# Autodesk Inventor assembly: BC-100001_B
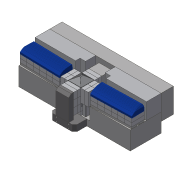
[picture p0: Inventor's stored thumbnail of the model, 180x180]
Saved by Autodesk Inventor 2016 (Build 200138000, 138)
## iProperties
Created: 2015-09-16
Part Number: BC-100001_B
Document SubType Name: Assembly
Designer: Reinaldo.Basílio
Author: Reinaldo.Basílio
## Documents named in this file (25)
- D:\ARQ\Basilio\LNLS-2\Anel\Dipolos\BC-3T\Dipolo 3T e 1T\Prototipo 1\Desenhos\BC-100001_B.iam
- D:\ARQ\Basilio\LNLS-2\Anel\Dipolos\BC-3T\Dipolo 3T e 1T\Prototipo 1\Desenhos\BC-100003.iam
- D:\ARQ\Basilio\LNLS-2\Anel\Dipolos\BC-3T\Dipolo 3T e 1T\Prototipo 1\Desenhos\BC-100004.iam
- D:\ARQ\Basilio\LNLS-2\Anel\Dipolos\BC-3T\Dipolo 3T e 1T\Prototipo 1\Desenhos\BC-10009.ipt
- D:\ARQ\Basilio\LNLS-2\Anel\Dipolos\BC-3T\Dipolo 3T e 1T\Prototipo 1\Desenhos\BC-100005.iam
- D:\ARQ\Basilio\LNLS-2\Anel\Dipolos\BC-3T\Dipolo 3T e 1T\Prototipo 1\Desenhos\BC-10010.ipt
- D:\ARQ\Basilio\LNLS-2\Anel\Dipolos\BC-3T\Dipolo 3T e 1T\Prototipo 1\Desenhos\BC-10011.ipt
- D:\ARQ\Basilio\LNLS-2\Anel\Dipolos\BC-3T\Dipolo 3T e 1T\Prototipo 1\Projeto Mecanico\BC-10001_B.ipt
- D:\ARQ\Basilio\LNLS-2\Anel\Dipolos\BC-3T\Dipolo 3T e 1T\Prototipo 1\Desenhos\BC-10012.ipt
- D:\ARQ\Basilio\LNLS-2\Anel\Dipolos\BC-3T\Dipolo 3T e 1T\Prototipo 1\Desenhos\BC-10002_C.ipt
- D:\ARQ\Basilio\LNLS-2\Anel\Dipolos\BC-3T\Dipolo 3T e 1T\Prototipo 1\Desenhos\BC-10013.ipt
- D:\ARQ\Basilio\LNLS-2\Anel\Dipolos\BC-3T\Dipolo 3T e 1T\Prototipo 1\Desenhos\BC-100014.ipt
- D:\ARQ\Basilio\LNLS-2\Anel\Dipolos\BC-3T\Dipolo 3T e 1T\Prototipo 1\Desenhos\BC-100003-B.iam
- D:\ARQ\Basilio\LNLS-2\Anel\Dipolos\BC-3T\Dipolo 3T e 1T\Prototipo 1\Desenhos\BC-100001_B\AIP\FEA\bjj5sjyio.fins
- D:\ARQ\Basilio\LNLS-2\Anel\Dipolos\BC-3T\Dipolo 3T e 1T\Prototipo 1\Desenhos\BC-100001_B\AIP\FEA\bjj5sjyio.fsat
- D:\ARQ\Basilio\LNLS-2\Anel\Dipolos\BC-3T\Dipolo 3T e 1T\Prototipo 1\Desenhos\BC-100001_B\AIP\FEA\bjj5sjyio.ftes
- D:\ARQ\Basilio\LNLS-2\Anel\Dipolos\BC-3T\Dipolo 3T e 1T\Prototipo 1\Desenhos\BC-100001_B\AIP\FEA\bjj5sjyio.fwiz
- D:\ARQ\Basilio\LNLS-2\Anel\Dipolos\BC-3T\Dipolo 3T e 1T\Prototipo 1\Desenhos\BC-100001_B\AIP\FEA\bjj5sjykg.fmsh
- D:\ARQ\Basilio\LNLS-2\Anel\Dipolos\BC-3T\Dipolo 3T e 1T\Prototipo 1\Desenhos\BC-100001_B\AIP\FEA\bjj5sjykh.fres
- D:\ARQ\Basilio\LNLS-2\Anel\Dipolos\BC-3T\Dipolo 3T e 1T\Prototipo 1\Desenhos\BC-100001_B\AIP\FEA\bkc5hc0u8.fins
- D:\ARQ\Basilio\LNLS-2\Anel\Dipolos\BC-3T\Dipolo 3T e 1T\Prototipo 1\Desenhos\BC-100001_B\AIP\FEA\bkc5hc0u8.fsat
- D:\ARQ\Basilio\LNLS-2\Anel\Dipolos\BC-3T\Dipolo 3T e 1T\Prototipo 1\Desenhos\BC-100001_B\AIP\FEA\bkc5hc0u8.ftes
- D:\ARQ\Basilio\LNLS-2\Anel\Dipolos\BC-3T\Dipolo 3T e 1T\Prototipo 1\Desenhos\BC-100001_B\AIP\FEA\bkc5hc0u8.fwiz
- D:\ARQ\Basilio\LNLS-2\Anel\Dipolos\BC-3T\Dipolo 3T e 1T\Prototipo 1\Desenhos\BC-100001_B\AIP\FEA\bkc5hc1c0.fmsh
- D:\ARQ\Basilio\LNLS-2\Anel\Dipolos\BC-3T\Dipolo 3T e 1T\Prototipo 1\Desenhos\BC-100001_B\AIP\FEA\bkc5hc1c1.fres
## Components (17 placed, 12 different names)
1. BC-10001_B:1 — Flush:36, Flush:41, Insert:1, Insert:2, Mate:36, Mate:39, Flush:47, Flush:49, Mate:46, Mate:47, Flush:50, Flush:51, Flush:52, Flush:53, Mate:48, Mate:50, Mate:52, Flush:57, Insert:3, Tangent:1, Insert:4, Tangent:2
2. BC-10002_C:1 — Flush:46, Mate:48, Mate:49
3. BC-100003-B:1 [sub-assembly] — Insert:3, Tangent:1
4. BC-100003:2 [sub-assembly] — Insert:4, Tangent:2
5. BC-100004:1 [sub-assembly] — Flush:24, Mate:17, Flush:25, Flush:26, Mate:50
6. BC-10009:1 — Mate:17, Flush:25, Flush:26, Mate:18, Flush:27, Flush:28, Mate:22, Flush:29, Mate:24, Flush:30, Mate:28, Flush:33, Mate:29, Flush:34, Mate:30, Flush:36, Flush:41, Flush:43, Mate:37, Mate:38, Mate:40, Mate:41, Flush:46
7. BC-100005:1 [sub-assembly] — Flush:28, Mate:30, Flush:35, Mate:49
8. BC-100005:2 [sub-assembly] — Mate:18, Flush:27, Flush:31, Flush:32, Flush:34
9. BC-100004:2 [sub-assembly] — Mate:22, Flush:29, Flush:31
10. BC-100004:3 [sub-assembly] — Mate:24, Flush:30, Flush:32, Flush:35
11. BC-10010:1 — Insert:1, Insert:2, Flush:42, Mate:34
12. BC-10011:1 — Flush:42, Mate:34, Flush:43
13. BC-10012:1 — Mate:36, Mate:37, Mate:38
14. BC-10012:2 — Mate:39, Mate:40, Mate:41
15. BC-10013:1 — Flush:49, Mate:47, Flush:50, Flush:53
16. BC-10013:2 — Flush:47, Mate:46, Flush:51, Flush:52, Flush:56
17. BC-100014:1 — Mate:52, Flush:56, Flush:57
## Relationships (51: Flush 25, Mate 20, Insert 4, Tangent 2)
- Flush:24: BC-100004:1
- Mate:17: BC-100004:1 ↔ BC-10009:1
- Flush:25: BC-100004:1 ↔ BC-10009:1
- Flush:26: BC-100004:1 ↔ BC-10009:1
- Mate:18: BC-10009:1 ↔ BC-100005:2
- Flush:27: BC-10009:1 ↔ BC-100005:2
- Flush:28: BC-10009:1 ↔ BC-100005:1
- Mate:22: BC-10009:1 ↔ BC-100004:2
- Flush:29: BC-10009:1 ↔ BC-100004:2
- Mate:24: BC-10009:1 ↔ BC-100004:3
- Flush:30: BC-10009:1 ↔ BC-100004:3
- Flush:31: BC-100005:2 ↔ BC-100004:2
- Flush:32: BC-100005:2 ↔ BC-100004:3
- Mate:28: BC-10009:1
- Flush:33: BC-10009:1
- Mate:29: BC-10009:1
- Flush:34 (-30 mm): BC-10009:1 ↔ BC-100005:2
- Mate:30: BC-10009:1 ↔ BC-100005:1
- Flush:35: BC-100005:1 ↔ BC-100004:3
- Flush:36: BC-10001_B:1 ↔ BC-10009:1
- Flush:41: BC-10001_B:1 ↔ BC-10009:1
- Insert:1: BC-10001_B:1 ↔ BC-10010:1
- Insert:2: BC-10001_B:1 ↔ BC-10010:1
- Flush:42: BC-10010:1 ↔ BC-10011:1
- Mate:34: BC-10010:1 ↔ BC-10011:1
- Flush:43: BC-10009:1 ↔ BC-10011:1
- Mate:36: BC-10001_B:1 ↔ BC-10012:1
- Mate:37: BC-10009:1 ↔ BC-10012:1
- Mate:38: BC-10009:1 ↔ BC-10012:1
- Mate:39: BC-10001_B:1 ↔ BC-10012:2
- Mate:40: BC-10009:1 ↔ BC-10012:2
- Mate:41: BC-10009:1 ↔ BC-10012:2
- Flush:46: BC-10002_C:1 ↔ BC-10009:1
- Flush:47: BC-10001_B:1 ↔ BC-10013:2
- Flush:49: BC-10001_B:1 ↔ BC-10013:1
- Mate:46: BC-10001_B:1 ↔ BC-10013:2
- Mate:47: BC-10001_B:1 ↔ BC-10013:1
- Flush:50: BC-10001_B:1 ↔ BC-10013:1
- Flush:51: BC-10001_B:1 ↔ BC-10013:2
- Flush:52: BC-10001_B:1 ↔ BC-10013:2
- Flush:53: BC-10001_B:1 ↔ BC-10013:1
- Mate:48: BC-10001_B:1 ↔ BC-10002_C:1
- Mate:49: BC-10002_C:1 ↔ BC-100005:1
- Mate:50: BC-10001_B:1 ↔ BC-100004:1
- Mate:52: BC-10001_B:1 ↔ BC-100014:1
- Flush:56: BC-10013:2 ↔ BC-100014:1
- Flush:57: BC-10001_B:1 ↔ BC-100014:1
- Insert:3: BC-10001_B:1 ↔ BC-100003-B:1
- Tangent:1: BC-10001_B:1 ↔ BC-100003-B:1
- Insert:4: BC-10001_B:1 ↔ BC-100003:2
- Tangent:2: BC-10001_B:1 ↔ BC-100003:2
## Named parameters: sa_0 = 0, sa_1 = -1.18424e-08, sa_2 = 5e+06, sa_3 = -0, sa_4 = -0, sa_5 = 5e+06
note: some values were not read from the file. Shown as the stored number, unit unknown: "sa_0", "sa_1", "sa_2", "sa_3", "sa_4", "sa_5".
